# Autodesk Inventor assembly: BAG Motor with 100-to-1 0.5in. Round Output Shaft
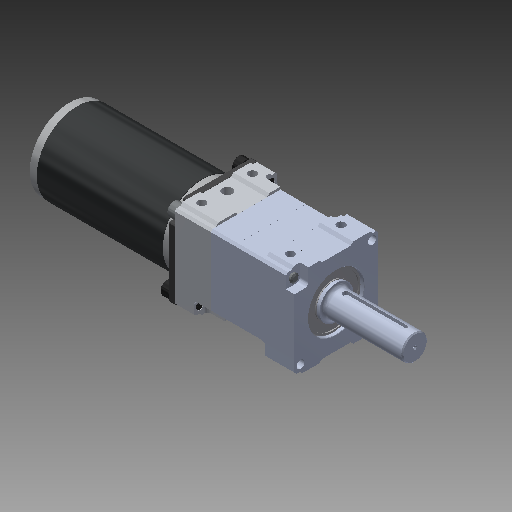
[picture p0: Inventor's stored thumbnail of the model, 512x512]
Saved by Autodesk Inventor 2019 (Build 230136000, 136)
## iProperties
Created: 2016-10-31
Part Number: BAG Motor with 100-to-1 0.5in. Round Output Shaft
Description: STEP AP214
Document SubType Name: Assembly
Designer: Alex Barnett
Sending System: SolidWorks 2016
Preprocessor: SwSTEP 2.0
Title: 217-4973_2stage_BAG.STEP
Revision Number: ANY
## Documents named in this file (17)
- C:\Users\Alex Barnett\Documents\Robotics '18-19\CAD\(2) Bucket Chain Lead Screw Design\Roller\Top Roller & Mounts - Copy\VEX Motors\BAG Motor with 100-to-1 0.5in. Round Output Shaft.iam
- C:\Users\Alex Barnett\Documents\Robotics '18-19\CAD\(2) Bucket Chain Lead Screw Design\Roller\Top Roller & Mounts - Copy\VEX Motors\217-2625-026 Rev1.ipt
- C:\Users\Alex Barnett\Documents\Robotics '18-19\CAD\(2) Bucket Chain Lead Screw Design\Roller\Top Roller & Mounts - Copy\VEX Motors\217-2742-001 Rev4.ipt
- C:\Users\Alex Barnett\Documents\Robotics '18-19\CAD\(2) Bucket Chain Lead Screw Design\Roller\Top Roller & Mounts - Copy\VEX Motors\217-2625-017 Rev1_9714K61.ipt
- C:\Users\Alex Barnett\Documents\Robotics '18-19\CAD\(2) Bucket Chain Lead Screw Design\Roller\Top Roller & Mounts - Copy\VEX Motors\217-2625-018 Rev1_98541A410.ipt
- C:\Users\Alex Barnett\Documents\Robotics '18-19\CAD\(2) Bucket Chain Lead Screw Design\Roller\Top Roller & Mounts - Copy\VEX Motors\832-2250-Base-Kit-Screw_SSA0832-0500ZC.ipt
- C:\Users\Alex Barnett\Documents\Robotics '18-19\CAD\(2) Bucket Chain Lead Screw Design\Roller\Top Roller & Mounts - Copy\VEX Motors\217-2625-025 Rev1.ipt
- C:\Users\Alex Barnett\Documents\Robotics '18-19\CAD\(2) Bucket Chain Lead Screw Design\Roller\Top Roller & Mounts - Copy\VEX Motors\217-4649-002 Rev1_SSA0832-0500ZC.ipt
- C:\Users\Alex Barnett\Documents\Robotics '18-19\CAD\(2) Bucket Chain Lead Screw Design\Roller\Top Roller & Mounts - Copy\VEX Motors\217-4649-006 Rev1_SSA0004-008BA.ipt
- C:\Users\Alex Barnett\Documents\Robotics '18-19\CAD\(2) Bucket Chain Lead Screw Design\Roller\Top Roller & Mounts - Copy\VEX Motors\217-2822-003 Rev4.ipt
- C:\Users\Alex Barnett\Documents\Robotics '18-19\CAD\(2) Bucket Chain Lead Screw Design\Roller\Top Roller & Mounts - Copy\VEX Motors\217-3351 Rev2.ipt
- C:\Users\Alex Barnett\Documents\Robotics '18-19\CAD\(2) Bucket Chain Lead Screw Design\Roller\Top Roller & Mounts - Copy\VEX Motors\217-2820 Rev1_Public.iam
- C:\Users\Alex Barnett\Documents\Robotics '18-19\CAD\(2) Bucket Chain Lead Screw Design\Roller\Top Roller & Mounts - Copy\VEX Motors\217-2816-001 Rev1.ipt
- C:\Users\Alex Barnett\Documents\Robotics '18-19\CAD\(2) Bucket Chain Lead Screw Design\Roller\Top Roller & Mounts - Copy\VEX Motors\217-4649-001 Rev1.ipt
- C:\Users\Alex Barnett\Documents\Robotics '18-19\CAD\(2) Bucket Chain Lead Screw Design\Roller\Top Roller & Mounts - Copy\VEX Motors\217-4649-007 Rev1_94105A824.ipt
- C:\Users\Alex Barnett\Documents\Robotics '18-19\CAD\(2) Bucket Chain Lead Screw Design\Roller\Top Roller & Mounts - Copy\VEX Motors\217-2625-011 Rev1.ipt
- C:\Users\Alex Barnett\Documents\Robotics '18-19\CAD\(2) Bucket Chain Lead Screw Design\Roller\Top Roller & Mounts - Copy\VEX Motors\VersaPlanetary 1-2in. Round Output Shaft.ipt
## Components (22 placed, 22 different names)
1. 217-2625-026 Rev1_1
2. 217-2742-001 Rev4_2
3. 217-2742-001 Rev4_3 — Mate:1, Mate:2
4. 217-2625-017 Rev1_9714K61_4
5. 217-2625-018 Rev1_98541A410_6
6. 832-2250-Base-Kit-Screw_SSA0832-0500ZC_7
7. 832-2250-Base-Kit-Screw_SSA0832-0500ZC_8
8. 217-2625-025 Rev1_9
9. 217-4649-002 Rev1_SSA0832-0500ZC_10
10. 217-4649-002 Rev1_SSA0832-0500ZC_11
11. 217-4649-006 Rev1_SSA0004-008BA_12
12. 217-4649-006 Rev1_SSA0004-008BA_13
13. 217-2822-003 Rev4_14
14. 217-3351 Rev2_15
15. 217-2820 Rev1_Public_16 [sub-assembly]
16. 217-2816-001 Rev1_17
17. 217-2820 Rev1_Public_18 [sub-assembly]
18. 217-2816-001 Rev1_19
19. 217-4649-001 Rev1_20
20. 217-4649-007 Rev1_94105A824_21
21. 217-2625-011 Rev1_22
22. VersaPlanetary 1-2in. Round Output Shaft:1 — Mate:1, Mate:2
## Relationships (2: Mate 2)
- Mate:1: 217-2742-001 Rev4_3 ↔ VersaPlanetary 1-2in. Round Output Shaft:1
- Mate:2: 217-2742-001 Rev4_3 ↔ VersaPlanetary 1-2in. Round Output Shaft:1
